(part 1 of 2)
# Autodesk Inventor assembly: Table
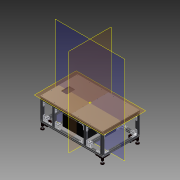
[picture p0: Inventor's stored thumbnail of the model, 180x180]
Saved by Autodesk Inventor 2015 (Build 190159000, 159)
## iProperties
Created: 2015-12-24
Part Number: Table
Document SubType Name: Assembly
Designer: Ryo
Author: Ryo
## Documents named in this file (11)
- D:\Users\Ryo\Documents\Inventor\motoman_cad\SIA5_TABLE\INVENTOR2015\Table.iam
- D:\Users\Ryo\Documents\Inventor\motoman_table\EFS8-4040-580.ipt
- D:\Users\Ryo\Documents\Inventor\motoman_table\EFS8-4040-305.ipt
- D:\Users\Ryo\Documents\Inventor\motoman_cad\SIA5_TABLE\parts\EFS8-4040-1100.ipt
- D:\Users\Ryo\Documents\Inventor\motoman_cad\SIA5_TABLE\parts\SFK-N19T.ipt
- D:\Users\Ryo\Documents\Inventor\motoman_cad\SIA5_TABLE\INVENTOR2015\board.ipt
- D:\Users\Ryo\Documents\Inventor\motoman_cad\SIA5_TABLE\INVENTOR2015\controller_table.ipt
- D:\Users\Ryo\Documents\Inventor\motoman_cad\SIA5_TABLE\INVENTOR2015\controller.ipt
- D:\Users\Ryo\Documents\Inventor\Content Center Files\R2015\ja-JP\JIS B 1176\JIS B 1176 - M8 x 12.ipt
- D:\Users\Ryo\Documents\Inventor\Content Center Files\R2015\ja-JP\JIS B 1176\JIS B 1176 - M6 x 10.ipt
- D:\Users\Ryo\Documents\Inventor\motoman_cad\SIA5_TABLE\INVENTOR2015\foot_parts.iam
## Components (309 placed, 10 different names)
1. EFS8-4040-580:1 — フラッシュ:63, フラッシュ:64, メイト:70, フラッシュ:82, メイト:81, メイト:85, メイト:89, フラッシュ:86, メイト:91, フラッシュ:114
2. EFS8-4040-580:2 — フラッシュ:43, フラッシュ:44, メイト:44, フラッシュ:47, メイト:47, フラッシュ:49, メイト:51, フラッシュ:83, メイト:83, フラッシュ:89, メイト:95, フラッシュ:119, フラッシュ:122
3. EFS8-4040-580:4 — フラッシュ:16, メイト:26, フラッシュ:17, フラッシュ:18, フラッシュ:20, フラッシュ:54, メイト:62, フラッシュ:77, フラッシュ:78, フラッシュ:98, メイト:114, メイト:116, メイト:133
4. EFS8-4040-580:5 — フラッシュ:74, フラッシュ:75, メイト:73, フラッシュ:76, フラッシュ:95, メイト:108, フラッシュ:96, メイト:109, フラッシュ:101, メイト:119, フラッシュ:102, メイト:121
5. EFS8-4040-580:6 — フラッシュ:1, メイト:14, フラッシュ:2, フラッシュ:3, メイト:15, フラッシュ:4, フラッシュ:13, メイト:20, フラッシュ:15, メイト:24, フラッシュ:74, メイト:112, フラッシュ:100, メイト:117, フラッシュ:116, メイト:308, フラッシュ:118, メイト:309
6. EFS8-4040-580:7 — フラッシュ:68, メイト:72, フラッシュ:76, メイト:135, メイト:138, フラッシュ:111, メイト:140, フラッシュ:112, メイト:142
7. EFS8-4040-580:8 — フラッシュ:45, フラッシュ:46, メイト:45, フラッシュ:48, メイト:49, メイト:58, フラッシュ:52, メイト:74, フラッシュ:90, メイト:98, フラッシュ:91, メイト:100
8. EFS8-4040-305:1 — フラッシュ:18, フラッシュ:19, メイト:27, メイト:63, メイト:64, メイト:66, メイト:101, メイト:104
9. EFS8-4040-305:2 — フラッシュ:5, フラッシュ:6, メイト:16, メイト:18, フラッシュ:11, メイト:21, メイト:105, メイト:107
10. EFS8-4040-305:3 — フラッシュ:20, フラッシュ:21, メイト:28, メイト:34, メイト:36, フラッシュ:104, メイト:125, フラッシュ:105, メイト:128, メイト:134, フラッシュ:108
11. EFS8-4040-305:4 — フラッシュ:28, フラッシュ:29, メイト:32, メイト:42, メイト:46, フラッシュ:61, メイト:69, フラッシュ:62, メイト:90, メイト:94
12. EFS8-4040-305:5 — フラッシュ:7, フラッシュ:8, フラッシュ:9, メイト:17, メイト:22, メイト:25, メイト:120, フラッシュ:103, メイト:124
13. EFS8-4040-305:6 — フラッシュ:24, フラッシュ:25, メイト:30, フラッシュ:45, メイト:57, メイト:59, メイト:60, メイト:79, メイト:87
14. EFS8-4040-305:7 — フラッシュ:26, フラッシュ:27, メイト:31, メイト:50, メイト:52, メイト:54, フラッシュ:59, フラッシュ:60, メイト:68, メイト:78, メイト:82
15. EFS8-4040-305:8 — フラッシュ:22, フラッシュ:23, メイト:29, メイト:38, メイト:39, メイト:48, メイト:129, メイト:132
16. EFS8-4040-1100:1 — フラッシュ:3, メイト:15, フラッシュ:4, フラッシュ:7, フラッシュ:8, フラッシュ:9, メイト:17, フラッシュ:14, メイト:23, メイト:26, フラッシュ:17, フラッシュ:21, メイト:28, フラッシュ:22, フラッシュ:23, メイト:29, フラッシュ:28, フラッシュ:29, メイト:32, フラッシュ:30, メイト:33, メイト:35, フラッシュ:31, フラッシュ:32, メイト:37, フラッシュ:33, メイト:40, フラッシュ:42, メイト:43, フラッシュ:43, フラッシュ:44, フラッシュ:46, メイト:45, メイト:96, メイト:99, フラッシュ:99, メイト:115, メイト:118, フラッシュ:117, フラッシュ:120, メイト:310
17. EFS8-4040-1100:2 — フラッシュ:61, メイト:69, フラッシュ:62, フラッシュ:63, フラッシュ:68, メイト:72, フラッシュ:87, メイト:92, フラッシュ:88, メイト:93, メイト:122, メイト:123, メイト:126, メイト:127, フラッシュ:106, メイト:130, フラッシュ:107, メイト:131, メイト:139, メイト:141, メイト:307
18. EFS8-4040-1100:3 — フラッシュ:59, フラッシュ:60, メイト:68, フラッシュ:64, メイト:70, フラッシュ:75, メイト:73, フラッシュ:80, メイト:77, フラッシュ:81, メイト:80, フラッシュ:84, メイト:84, フラッシュ:85, メイト:88, フラッシュ:92, メイト:102, フラッシュ:93, メイト:103, フラッシュ:94, メイト:106, メイト:110, フラッシュ:109, メイト:136, フラッシュ:110, メイト:137, フラッシュ:113, メイト:313
19. EFS8-4040-1100:4 — フラッシュ:1, メイト:14, フラッシュ:2, フラッシュ:5, フラッシュ:6, メイト:16, フラッシュ:12, メイト:19, フラッシュ:16, フラッシュ:19, メイト:27, フラッシュ:24, フラッシュ:25, メイト:30, フラッシュ:26, フラッシュ:27, メイト:31, メイト:44, メイト:53, フラッシュ:51, メイト:56, フラッシュ:53, メイト:61, フラッシュ:55, メイト:65, フラッシュ:56, フラッシュ:57, メイト:67, フラッシュ:58, メイト:75, フラッシュ:79, メイト:86, メイト:97, フラッシュ:97, メイト:111, メイト:113, フラッシュ:115, フラッシュ:121, メイト:311
20. SFK-N19T:1 — フラッシュ:42, メイト:42, メイト:43, 挿入:1, 挿入:2, メイト:175, メイト:176, メイト:177, メイト:178
21. SFK-N19T:2 — フラッシュ:53, メイト:60, メイト:61, メイト:239, メイト:240, メイト:241, メイト:242, 挿入:15, 挿入:16
22. SFK-N19T:3 — フラッシュ:54, メイト:62, メイト:63, 挿入:79, 挿入:80, メイト:303, メイト:304, メイト:305, メイト:306
23. SFK-N19T:4 — フラッシュ:47, メイト:46, メイト:47, 挿入:5, 挿入:6, メイト:179, メイト:180, メイト:181, メイト:182
24. SFK-N19T:5 — フラッシュ:49, メイト:50, メイト:51, メイト:52, 挿入:7, 挿入:8, 挿入:19, 挿入:20
25. SFK-N19T:6 — メイト:58, フラッシュ:52, メイト:59, メイト:243, メイト:244, メイト:245, メイト:246, 挿入:23, 挿入:24
26. SFK-N19T:7 — フラッシュ:33, メイト:39, メイト:40, メイト:143, メイト:144, メイト:145, メイト:146, メイト:147, メイト:148, メイト:149, メイト:150
27. SFK-N19T:8 — メイト:35, フラッシュ:31, メイト:36, 挿入:45, 挿入:46, 挿入:55, 挿入:56
28. SFK-N19T:9 — フラッシュ:51, メイト:56, メイト:57, メイト:231, メイト:232, メイト:233, メイト:234, メイト:255, メイト:256, メイト:257, メイト:258
29. SFK-N19T:10 — フラッシュ:13, メイト:20, メイト:21, メイト:291, メイト:292, メイト:293, メイト:294, 挿入:115, 挿入:116
30. SFK-N19T:11 — メイト:53, メイト:54, フラッシュ:58, メイト:223, メイト:224, メイト:225, メイト:226, メイト:227, メイト:228, メイト:229, メイト:230
31. SFK-N19T:12 — フラッシュ:48, メイト:48, メイト:49, メイト:155, メイト:156, メイト:157, メイト:158, 挿入:113, 挿入:114
32. SFK-N19T:13 — フラッシュ:32, メイト:37, メイト:38, メイト:151, メイト:152, メイト:153, メイト:154, メイト:275, メイト:276, メイト:277, メイト:278
33. SFK-N19T:14 — フラッシュ:30, メイト:33, メイト:34, 挿入:37, 挿入:38, 挿入:57, 挿入:58
34. SFK-N19T:15 — メイト:18, フラッシュ:11, フラッシュ:12, メイト:19, メイト:287, メイト:288, メイト:289, メイト:290, 挿入:103, 挿入:104
35. SFK-N19T:16 — フラッシュ:15, メイト:24, メイト:25, 挿入:67, 挿入:68, 挿入:75, 挿入:76
36. SFK-N19T:17 — フラッシュ:55, メイト:64, メイト:65, 挿入:77, 挿入:78, 挿入:89, 挿入:90
37. SFK-N19T:18 — フラッシュ:14, メイト:22, メイト:23, 挿入:59, 挿入:60, 挿入:61, 挿入:62
38. SFK-N19T:19 — フラッシュ:56
39. SFK-N19T:20 — フラッシュ:57, メイト:66, メイト:67, 挿入:81, 挿入:82, 挿入:87, 挿入:88
40. board:1 — メイト:307, フラッシュ:113, フラッシュ:114, 挿入:125, 挿入:126, 挿入:127, 挿入:128, 挿入:129, 挿入:130, 挿入:131, 挿入:132, 挿入:133, 挿入:134, 挿入:135, 挿入:136, 挿入:137, 挿入:138, 挿入:139, 挿入:140, 挿入:141, 挿入:142, 挿入:143, 挿入:144, 挿入:145, 挿入:146, メイト:312, フラッシュ:123
41. controller_table:1 — メイト:74, メイト:75, フラッシュ:77, メイト:76
42. controller:1 — メイト:76, フラッシュ:78, フラッシュ:79
43. SFK-N19T:21 — フラッシュ:80, メイト:77, メイト:78, メイト:219, メイト:220, メイト:221, メイト:222, メイト:263, メイト:264, メイト:265, メイト:266
44. SFK-N19T:22 — フラッシュ:95, メイト:107, メイト:108, メイト:295, メイト:296, メイト:297, メイト:298, 挿入:123, 挿入:124
45. SFK-N19T:23 — フラッシュ:82, メイト:81, メイト:82, 挿入:17, 挿入:18, メイト:267, メイト:268, メイト:269, メイト:270
46. SFK-N19T:24 — フラッシュ:81, メイト:79, メイト:80, メイト:259, メイト:260, メイト:261, メイト:262, 挿入:25, 挿入:26
47. SFK-N19T:25 — フラッシュ:84, メイト:84, メイト:85, 挿入:13, 挿入:14, メイト:247, メイト:248, メイト:249, メイト:250
48. SFK-N19T:26 — フラッシュ:89, メイト:95, メイト:96, メイト:171, メイト:172, メイト:173, メイト:174, メイト:183, メイト:184, メイト:185, メイト:186
49. SFK-N19T:27 — フラッシュ:96, メイト:109, メイト:110, 挿入:99, 挿入:100, 挿入:117, 挿入:118
50. SFK-N19T:28 — フラッシュ:94, メイト:105, メイト:106, 挿入:97, 挿入:98, 挿入:101, 挿入:102
51. SFK-N19T:29 — フラッシュ:88, メイト:93, メイト:94, メイト:195, メイト:196, メイト:197, メイト:198, 挿入:33, 挿入:34
52. SFK-N19T:30 — メイト:89, フラッシュ:86, メイト:90, メイト:199, メイト:200, メイト:201, メイト:202, 挿入:29, 挿入:30
53. SFK-N19T:31 — フラッシュ:93, メイト:103, メイト:104, 挿入:91, 挿入:92, 挿入:93, 挿入:94
54. SFK-N19T:32 — フラッシュ:83, メイト:83, メイト:86, メイト:235, メイト:236, メイト:237, メイト:238, 挿入:21, 挿入:22
55. SFK-N19T:33 — フラッシュ:85, メイト:87, メイト:88, メイト:215, メイト:216, メイト:217, メイト:218, メイト:314, メイト:315, メイト:316, メイト:317
56. SFK-N19T:34 — フラッシュ:87, メイト:91, メイト:92, メイト:187, メイト:188, メイト:189, メイト:190, メイト:191, メイト:192, メイト:193, メイト:194
57. SFK-N19T:35 — フラッシュ:90, メイト:97, メイト:98, メイト:163, メイト:164, メイト:165, メイト:166, メイト:251, メイト:252, メイト:253, メイト:254
58. SFK-N19T:36 — フラッシュ:91, メイト:99, メイト:100, 挿入:3, 挿入:4, メイト:167, メイト:168, メイト:169, メイト:170
59. SFK-N19T:37 — フラッシュ:92, メイト:101, メイト:102, 挿入:83, 挿入:84, 挿入:95, 挿入:96
60. SFK-N19T:38 — フラッシュ:106, メイト:129, メイト:130, 挿入:9, 挿入:10, メイト:271, メイト:272, メイト:273, メイト:274
61. SFK-N19T:39 — フラッシュ:101, メイト:119, メイト:120, 挿入:69, 挿入:70, 挿入:71, 挿入:72
62. SFK-N19T:40 — フラッシュ:103, メイト:123, メイト:124, 挿入:49, 挿入:50, 挿入:51, 挿入:52
63. SFK-N19T:43 — メイト:139, フラッシュ:111, メイト:140, メイト:203, メイト:204, メイト:205, メイト:206, メイト:207, メイト:208, メイト:209, メイト:210
64. SFK-N19T:44 — フラッシュ:109, メイト:135, メイト:136, メイト:211, メイト:212, メイト:213, メイト:214, 挿入:119, 挿入:120
65. SFK-N19T:45 — フラッシュ:107, メイト:131, メイト:132, メイト:159, メイト:160, メイト:161, メイト:162, 挿入:31, 挿入:32
66. SFK-N19T:46 — フラッシュ:104, メイト:125, メイト:126, 挿入:39, 挿入:40, 挿入:41, 挿入:42
67. SFK-N19T:47 — フラッシュ:99, メイト:115, メイト:116, 挿入:43, 挿入:44, 挿入:65, 挿入:66
68. SFK-N19T:48 — フラッシュ:97, メイト:111, メイト:112, 挿入:105, 挿入:106, 挿入:107, 挿入:108
69. SFK-N19T:49 — フラッシュ:105, メイト:127, メイト:128, 挿入:35, 挿入:36, 挿入:47, 挿入:48
70. SFK-N19T:50 — フラッシュ:110, メイト:137, メイト:138, 挿入:27, 挿入:28, 挿入:121, 挿入:122
71. SFK-N19T:51 — メイト:133, メイト:134, フラッシュ:108, 挿入:63, 挿入:64, メイト:279, メイト:280, メイト:281, メイト:282
72. SFK-N19T:52 — フラッシュ:102, メイト:121, メイト:122, 挿入:73, 挿入:74, 挿入:111, 挿入:112
73. SFK-N19T:53 — フラッシュ:98, メイト:113, メイト:114, 挿入:85, 挿入:86, メイト:299, メイト:300, メイト:301, メイト:302
74. SFK-N19T:55 — フラッシュ:100, メイト:117, メイト:118, メイト:283, メイト:284, メイト:285, メイト:286, 挿入:109, 挿入:110
75. SFK-N19T:56 — フラッシュ:112, メイト:141, メイト:142, 挿入:11, 挿入:12, 挿入:53, 挿入:54
76. JIS B 1176 - メートル M8 x 12:1 — メイト:143, メイト:144
77. JIS B 1176 - メートル M8 x 12:2 — メイト:145, メイト:146
78. JIS B 1176 - メートル M8 x 12:3 — 挿入:1
79. JIS B 1176 - メートル M8 x 12:4 — 挿入:2
80. JIS B 1176 - メートル M8 x 12:5 — メイト:147, メイト:148
81. JIS B 1176 - メートル M8 x 12:6 — メイト:149, メイト:150
82. JIS B 1176 - メートル M8 x 12:7 — メイト:151, メイト:152
83. JIS B 1176 - メートル M8 x 12:8 — メイト:153, メイト:154
84. JIS B 1176 - メートル M8 x 12:9 — メイト:155, メイト:156
85. JIS B 1176 - メートル M8 x 12:10 — メイト:157, メイト:158
86. JIS B 1176 - メートル M8 x 12:11 — 挿入:3
87. JIS B 1176 - メートル M8 x 12:12 — 挿入:4
88. JIS B 1176 - メートル M8 x 12:13 — メイト:159, メイト:160
89. JIS B 1176 - メートル M8 x 12:14 — メイト:161, メイト:162
90. JIS B 1176 - メートル M8 x 12:15 — 挿入:5
91. JIS B 1176 - メートル M8 x 12:16 — 挿入:6
92. JIS B 1176 - メートル M8 x 12:17 — メイト:163, メイト:164
93. JIS B 1176 - メートル M8 x 12:18 — メイト:165, メイト:166
94. JIS B 1176 - メートル M8 x 12:19 — 挿入:7
95. JIS B 1176 - メートル M8 x 12:20 — 挿入:8
96. JIS B 1176 - メートル M8 x 12:21 — メイト:167, メイト:168
97. JIS B 1176 - メートル M8 x 12:22 — メイト:169, メイト:170
98. JIS B 1176 - メートル M8 x 12:23 — メイト:171, メイト:172
99. JIS B 1176 - メートル M8 x 12:24 — メイト:173, メイト:174
100. JIS B 1176 - メートル M8 x 12:25 — メイト:175, メイト:176
101. JIS B 1176 - メートル M8 x 12:26 — メイト:177, メイト:178
102. JIS B 1176 - メートル M8 x 12:27 — メイト:179, メイト:180
103. JIS B 1176 - メートル M8 x 12:28 — メイト:181, メイト:182
104. JIS B 1176 - メートル M8 x 12:29 — メイト:183, メイト:184
105. JIS B 1176 - メートル M8 x 12:30 — メイト:185, メイト:186
106. JIS B 1176 - メートル M8 x 12:31 — メイト:187, メイト:188
107. JIS B 1176 - メートル M8 x 12:32 — メイト:189, メイト:190
108. JIS B 1176 - メートル M8 x 12:33 — メイト:191, メイト:192
109. JIS B 1176 - メートル M8 x 12:34 — メイト:193, メイト:194
110. JIS B 1176 - メートル M8 x 12:35 — メイト:195, メイト:196
111. JIS B 1176 - メートル M8 x 12:36 — メイト:197, メイト:198
112. JIS B 1176 - メートル M8 x 12:37 — メイト:199, メイト:200
113. JIS B 1176 - メートル M8 x 12:38 — メイト:201, メイト:202
114. JIS B 1176 - メートル M8 x 12:39 — 挿入:9
115. JIS B 1176 - メートル M8 x 12:40 — 挿入:10
116. JIS B 1176 - メートル M8 x 12:41 — 挿入:11
117. JIS B 1176 - メートル M8 x 12:42 — 挿入:12
118. JIS B 1176 - メートル M8 x 12:43 — メイト:203, メイト:204
119. JIS B 1176 - メートル M8 x 12:44 — メイト:205, メイト:206
120. JIS B 1176 - メートル M8 x 12:45 — メイト:207, メイト:208
121. JIS B 1176 - メートル M8 x 12:46 — メイト:209, メイト:210
122. JIS B 1176 - メートル M8 x 12:47 — メイト:211, メイト:212
123. JIS B 1176 - メートル M8 x 12:48 — メイト:213, メイト:214
124. JIS B 1176 - メートル M8 x 12:49 — 挿入:13
125. JIS B 1176 - メートル M8 x 12:50 — 挿入:14
126. JIS B 1176 - メートル M8 x 12:51 — メイト:215, メイト:216
127. JIS B 1176 - メートル M8 x 12:52 — メイト:217, メイト:218
128. JIS B 1176 - メートル M8 x 12:53 — メイト:219, メイト:220
129. JIS B 1176 - メートル M8 x 12:54 — メイト:221, メイト:222
130. JIS B 1176 - メートル M8 x 12:55 — メイト:223, メイト:224
131. JIS B 1176 - メートル M8 x 12:56 — メイト:225, メイト:226
132. JIS B 1176 - メートル M8 x 12:57 — メイト:227, メイト:228
133. JIS B 1176 - メートル M8 x 12:58 — メイト:229, メイト:230
134. JIS B 1176 - メートル M8 x 12:59 — メイト:231, メイト:232
135. JIS B 1176 - メートル M8 x 12:60 — メイト:233, メイト:234
136. JIS B 1176 - メートル M8 x 12:61 — メイト:235, メイト:236
137. JIS B 1176 - メートル M8 x 12:62 — メイト:237, メイト:238
138. JIS B 1176 - メートル M8 x 12:63 — メイト:239, メイト:240
139. JIS B 1176 - メートル M8 x 12:64 — メイト:241, メイト:242
140. JIS B 1176 - メートル M8 x 12:65 — メイト:243, メイト:244
141. JIS B 1176 - メートル M8 x 12:66 — メイト:245, メイト:246
142. JIS B 1176 - メートル M8 x 12:67 — 挿入:15
143. JIS B 1176 - メートル M8 x 12:68 — 挿入:16
144. JIS B 1176 - メートル M8 x 12:69 — 挿入:17
145. JIS B 1176 - メートル M8 x 12:70 — 挿入:18
146. JIS B 1176 - メートル M8 x 12:71 — メイト:247, メイト:248
147. JIS B 1176 - メートル M8 x 12:72 — メイト:249, メイト:250
148. JIS B 1176 - メートル M8 x 12:73 — 挿入:19
149. JIS B 1176 - メートル M8 x 12:74 — 挿入:20
150. JIS B 1176 - メートル M8 x 12:75 — 挿入:21
151. JIS B 1176 - メートル M8 x 12:76 — 挿入:22
152. JIS B 1176 - メートル M8 x 12:77 — メイト:251, メイト:252
153. JIS B 1176 - メートル M8 x 12:78 — メイト:253, メイト:254
154. JIS B 1176 - メートル M8 x 12:79 — 挿入:23
155. JIS B 1176 - メートル M8 x 12:80 — 挿入:24
156. JIS B 1176 - メートル M8 x 12:81 — メイト:255, メイト:256
157. JIS B 1176 - メートル M8 x 12:82 — メイト:257, メイト:258
158. JIS B 1176 - メートル M8 x 12:83 — メイト:259, メイト:260
159. JIS B 1176 - メートル M8 x 12:84 — メイト:261, メイト:262
160. JIS B 1176 - メートル M8 x 12:85 — 挿入:25
161. JIS B 1176 - メートル M8 x 12:86 — 挿入:26
162. JIS B 1176 - メートル M8 x 12:87 — メイト:263, メイト:264
163. JIS B 1176 - メートル M8 x 12:88 — メイト:265, メイト:266
164. JIS B 1176 - メートル M8 x 12:89 — メイト:267, メイト:268
165. JIS B 1176 - メートル M8 x 12:90 — メイト:269, メイト:270
166. JIS B 1176 - メートル M8 x 12:91 — 挿入:27
167. JIS B 1176 - メートル M8 x 12:92 — 挿入:28
168. JIS B 1176 - メートル M8 x 12:93 — 挿入:29
169. JIS B 1176 - メートル M8 x 12:94 — 挿入:30
170. JIS B 1176 - メートル M8 x 12:95 — 挿入:31
171. JIS B 1176 - メートル M8 x 12:96 — 挿入:32
172. JIS B 1176 - メートル M8 x 12:97 — 挿入:33
173. JIS B 1176 - メートル M8 x 12:98 — 挿入:34
174. JIS B 1176 - メートル M8 x 12:99 — メイト:271, メイト:272
175. JIS B 1176 - メートル M8 x 12:100 — メイト:273, メイト:274
176. JIS B 1176 - メートル M8 x 12:101 — メイト:275, メイト:276
177. JIS B 1176 - メートル M8 x 12:102 — メイト:277, メイト:278
178. JIS B 1176 - メートル M8 x 12:103 — 挿入:35
179. JIS B 1176 - メートル M8 x 12:104 — 挿入:36
180. JIS B 1176 - メートル M8 x 12:105 — 挿入:37
181. JIS B 1176 - メートル M8 x 12:106 — 挿入:38
182. JIS B 1176 - メートル M8 x 12:107 — 挿入:39
183. JIS B 1176 - メートル M8 x 12:108 — 挿入:40
184. JIS B 1176 - メートル M8 x 12:109 — 挿入:41
185. JIS B 1176 - メートル M8 x 12:110 — 挿入:42
186. JIS B 1176 - メートル M8 x 12:111 — 挿入:43
187. JIS B 1176 - メートル M8 x 12:112 — 挿入:44
188. JIS B 1176 - メートル M8 x 12:113 — 挿入:45
189. JIS B 1176 - メートル M8 x 12:114 — 挿入:46
190. JIS B 1176 - メートル M8 x 12:115 — 挿入:47
191. JIS B 1176 - メートル M8 x 12:116 — 挿入:48
192. JIS B 1176 - メートル M8 x 12:117 — 挿入:49
193. JIS B 1176 - メートル M8 x 12:118 — 挿入:50
194. JIS B 1176 - メートル M8 x 12:119 — 挿入:51
195. JIS B 1176 - メートル M8 x 12:120 — 挿入:52
196. JIS B 1176 - メートル M8 x 12:121 — 挿入:53
197. JIS B 1176 - メートル M8 x 12:122 — 挿入:54
198. JIS B 1176 - メートル M8 x 12:123 — 挿入:55
199. JIS B 1176 - メートル M8 x 12:124 — 挿入:56
200. JIS B 1176 - メートル M8 x 12:125 — 挿入:57
201. JIS B 1176 - メートル M8 x 12:126 — 挿入:58
202. JIS B 1176 - メートル M8 x 12:127 — 挿入:59
203. JIS B 1176 - メートル M8 x 12:128 — 挿入:60
204. JIS B 1176 - メートル M8 x 12:129 — 挿入:61
205. JIS B 1176 - メートル M8 x 12:130 — 挿入:62
206. JIS B 1176 - メートル M8 x 12:131 — 挿入:63
207. JIS B 1176 - メートル M8 x 12:132 — 挿入:64
208. JIS B 1176 - メートル M8 x 12:133 — 挿入:65
209. JIS B 1176 - メートル M8 x 12:134 — 挿入:66
210. JIS B 1176 - メートル M8 x 12:135 — 挿入:67
211. JIS B 1176 - メートル M8 x 12:136 — 挿入:68
212. JIS B 1176 - メートル M8 x 12:137 — 挿入:69
213. JIS B 1176 - メートル M8 x 12:138 — 挿入:70
214. JIS B 1176 - メートル M8 x 12:139 — 挿入:71
215. JIS B 1176 - メートル M8 x 12:140 — 挿入:72
216. JIS B 1176 - メートル M8 x 12:141 — 挿入:73
217. JIS B 1176 - メートル M8 x 12:142 — 挿入:74
218. JIS B 1176 - メートル M8 x 12:143 — メイト:279, メイト:280
219. JIS B 1176 - メートル M8 x 12:144 — メイト:281, メイト:282
220. JIS B 1176 - メートル M8 x 12:145 — 挿入:75
221. JIS B 1176 - メートル M8 x 12:146 — 挿入:76
222. JIS B 1176 - メートル M8 x 12:147 — メイト:283, メイト:284
223. JIS B 1176 - メートル M8 x 12:148 — メイト:285, メイト:286
224. JIS B 1176 - メートル M8 x 12:149 — 挿入:77
225. JIS B 1176 - メートル M8 x 12:150 — 挿入:78
226. JIS B 1176 - メートル M8 x 12:151 — 挿入:79
227. JIS B 1176 - メートル M8 x 12:152 — 挿入:80
228. JIS B 1176 - メートル M8 x 12:153 — 挿入:81
229. JIS B 1176 - メートル M8 x 12:154 — 挿入:82
230. JIS B 1176 - メートル M8 x 12:155 — 挿入:83
231. JIS B 1176 - メートル M8 x 12:156 — 挿入:84
232. JIS B 1176 - メートル M8 x 12:157 — 挿入:85
233. JIS B 1176 - メートル M8 x 12:158 — 挿入:86
234. JIS B 1176 - メートル M8 x 12:159 — 挿入:87
235. JIS B 1176 - メートル M8 x 12:160 — 挿入:88
236. JIS B 1176 - メートル M8 x 12:161 — メイト:287, メイト:288
237. JIS B 1176 - メートル M8 x 12:162 — メイト:289, メイト:290
238. JIS B 1176 - メートル M8 x 12:163 — メイト:291, メイト:292
239. JIS B 1176 - メートル M8 x 12:164 — メイト:293, メイト:294
240. JIS B 1176 - メートル M8 x 12:165 — 挿入:89
241. JIS B 1176 - メートル M8 x 12:166 — 挿入:90
242. JIS B 1176 - メートル M8 x 12:167 — 挿入:91
243. JIS B 1176 - メートル M8 x 12:168 — 挿入:92
244. JIS B 1176 - メートル M8 x 12:169 — 挿入:93
245. JIS B 1176 - メートル M8 x 12:170 — 挿入:94
246. JIS B 1176 - メートル M8 x 12:171 — 挿入:95
247. JIS B 1176 - メートル M8 x 12:172 — 挿入:96
248. JIS B 1176 - メートル M8 x 12:173 — 挿入:97
249. JIS B 1176 - メートル M8 x 12:174 — 挿入:98
250. JIS B 1176 - メートル M8 x 12:175 — 挿入:99
251. JIS B 1176 - メートル M8 x 12:176 — 挿入:100
252. JIS B 1176 - メートル M8 x 12:177 — メイト:295, メイト:296
253. JIS B 1176 - メートル M8 x 12:178 — メイト:297, メイト:298
254. JIS B 1176 - メートル M8 x 12:179 — 挿入:101
255. JIS B 1176 - メートル M8 x 12:180 — 挿入:102
256. JIS B 1176 - メートル M8 x 12:181 — 挿入:103
257. JIS B 1176 - メートル M8 x 12:182 — 挿入:104
258. JIS B 1176 - メートル M8 x 12:183 — 挿入:105
259. JIS B 1176 - メートル M8 x 12:184 — 挿入:106
260. JIS B 1176 - メートル M8 x 12:185 — 挿入:107
261. JIS B 1176 - メートル M8 x 12:186 — 挿入:108
262. JIS B 1176 - メートル M8 x 12:187 — メイト:299, メイト:300
263. JIS B 1176 - メートル M8 x 12:188 — メイト:301, メイト:302
264. JIS B 1176 - メートル M8 x 12:189 — 挿入:109
265. JIS B 1176 - メートル M8 x 12:190 — 挿入:110
266. JIS B 1176 - メートル M8 x 12:191 — 挿入:111
267. JIS B 1176 - メートル M8 x 12:192 — 挿入:112
268. JIS B 1176 - メートル M8 x 12:193 — 挿入:113
269. JIS B 1176 - メートル M8 x 12:194 — 挿入:114
270. JIS B 1176 - メートル M8 x 12:195 — メイト:303, メイト:304
271. JIS B 1176 - メートル M8 x 12:196 — メイト:305, メイト:306
272. JIS B 1176 - メートル M8 x 12:197 — 挿入:115
273. JIS B 1176 - メートル M8 x 12:198 — 挿入:116
274. JIS B 1176 - メートル M8 x 12:199 — 挿入:117
275. JIS B 1176 - メートル M8 x 12:200 — 挿入:118
276. JIS B 1176 - メートル M8 x 12:201 — 挿入:119
277. JIS B 1176 - メートル M8 x 12:202 — 挿入:120
278. JIS B 1176 - メートル M8 x 12:203 — 挿入:121
279. JIS B 1176 - メートル M8 x 12:204 — 挿入:122
280. JIS B 1176 - メートル M8 x 12:205 — 挿入:123
281. JIS B 1176 - メートル M8 x 12:206 — 挿入:124
282. JIS B 1176 - メートル M6 x 10:1 — 挿入:125
283. JIS B 1176 - メートル M6 x 10:2 — 挿入:126
284. JIS B 1176 - メートル M6 x 10:3 — 挿入:127
285. JIS B 1176 - メートル M6 x 10:4 — 挿入:128
286. JIS B 1176 - メートル M6 x 10:5 — 挿入:129
287. JIS B 1176 - メートル M6 x 10:6 — 挿入:130
288. JIS B 1176 - メートル M6 x 10:7 — 挿入:131
289. JIS B 1176 - メートル M6 x 10:8 — 挿入:132
290. JIS B 1176 - メートル M6 x 10:9 — 挿入:133
291. JIS B 1176 - メートル M6 x 10:10 — 挿入:134
292. JIS B 1176 - メートル M6 x 10:11 — 挿入:135
293. JIS B 1176 - メートル M6 x 10:12 — 挿入:136
294. JIS B 1176 - メートル M6 x 10:13 — 挿入:137
295. JIS B 1176 - メートル M6 x 10:14 — 挿入:138
296. JIS B 1176 - メートル M6 x 10:15 — 挿入:139
297. JIS B 1176 - メートル M6 x 10:16 — 挿入:140
298. JIS B 1176 - メートル M6 x 10:17 — 挿入:141
299. JIS B 1176 - メートル M6 x 10:18 — 挿入:142
300. JIS B 1176 - メートル M6 x 10:19 — 挿入:143
301. JIS B 1176 - メートル M6 x 10:20 — 挿入:144
302. JIS B 1176 - メートル M6 x 10:21 — 挿入:145
303. JIS B 1176 - メートル M6 x 10:22 — 挿入:146
304. foot_parts:1 [sub-assembly] — フラッシュ:115, フラッシュ:116, メイト:308
305. foot_parts:2 [sub-assembly] — フラッシュ:117, フラッシュ:118, メイト:309
306. foot_parts:3 [sub-assembly] — フラッシュ:119, フラッシュ:120, メイト:310
307. foot_parts:4 [sub-assembly] — フラッシュ:121, フラッシュ:122, メイト:311
308. JIS B 1176 - メートル M8 x 12:207 — メイト:314, メイト:315
309. JIS B 1176 - メートル M8 x 12:208 — メイト:316, メイト:317
## Relationships (552: Mate 301, Insert 146, Flush 105)
- フラッシュ:1 [Flush]: EFS8-4040-580:6 ↔ EFS8-4040-1100:4
- メイト:14 [Mate]: EFS8-4040-580:6 ↔ EFS8-4040-1100:4
- フラッシュ:2 [Flush]: EFS8-4040-580:6 ↔ EFS8-4040-1100:4
- フラッシュ:3 [Flush]: EFS8-4040-580:6 ↔ EFS8-4040-1100:1
- メイト:15 [Mate]: EFS8-4040-580:6 ↔ EFS8-4040-1100:1
- フラッシュ:4 [Flush]: EFS8-4040-580:6 ↔ EFS8-4040-1100:1
- フラッシュ:5 [Flush]: EFS8-4040-305:2 ↔ EFS8-4040-1100:4
- フラッシュ:6 [Flush]: EFS8-4040-305:2 ↔ EFS8-4040-1100:4
- メイト:16 [Mate]: EFS8-4040-305:2 ↔ EFS8-4040-1100:4
- フラッシュ:7 [Flush]: EFS8-4040-305:5 ↔ EFS8-4040-1100:1
- フラッシュ:8 [Flush]: EFS8-4040-305:5 ↔ EFS8-4040-1100:1
- フラッシュ:9 [Flush]: EFS8-4040-305:5 ↔ EFS8-4040-1100:1
- メイト:17 [Mate]: EFS8-4040-305:5 ↔ EFS8-4040-1100:1
- メイト:18 [Mate]: EFS8-4040-305:2 ↔ SFK-N19T:15
- フラッシュ:11 [Flush] (5 mm): EFS8-4040-305:2 ↔ SFK-N19T:15
- フラッシュ:12 [Flush] (5 mm): EFS8-4040-1100:4 ↔ SFK-N19T:15
- メイト:19 [Mate]: EFS8-4040-1100:4 ↔ SFK-N19T:15
- フラッシュ:13 [Flush] (5 mm): EFS8-4040-580:6 ↔ SFK-N19T:10
- メイト:20 [Mate]: EFS8-4040-580:6 ↔ SFK-N19T:10
- メイト:21 [Mate]: EFS8-4040-305:2 ↔ SFK-N19T:10
- フラッシュ:14 [Flush] (5 mm): EFS8-4040-1100:1 ↔ SFK-N19T:18
- メイト:22 [Mate]: EFS8-4040-305:5 ↔ SFK-N19T:18
- メイト:23 [Mate]: EFS8-4040-1100:1 ↔ SFK-N19T:18
- フラッシュ:15 [Flush] (5 mm): EFS8-4040-580:6 ↔ SFK-N19T:16
- メイト:24 [Mate]: EFS8-4040-580:6 ↔ SFK-N19T:16
- メイト:25 [Mate]: EFS8-4040-305:5 ↔ SFK-N19T:16
- フラッシュ:16 [Flush] (295 mm): EFS8-4040-580:4 ↔ EFS8-4040-1100:4
- メイト:26 [Mate]: EFS8-4040-580:4 ↔ EFS8-4040-1100:1
- フラッシュ:17 [Flush]: EFS8-4040-580:4 ↔ EFS8-4040-1100:1
- フラッシュ:18 [Flush]: EFS8-4040-580:4 ↔ EFS8-4040-305:1
- フラッシュ:19 [Flush]: EFS8-4040-305:1 ↔ EFS8-4040-1100:4
- メイト:27 [Mate]: EFS8-4040-305:1 ↔ EFS8-4040-1100:4
- フラッシュ:20 [Flush]: EFS8-4040-580:4 ↔ EFS8-4040-305:3
- フラッシュ:21 [Flush]: EFS8-4040-305:3 ↔ EFS8-4040-1100:1
- メイト:28 [Mate]: EFS8-4040-305:3 ↔ EFS8-4040-1100:1
- フラッシュ:22 [Flush] (210 mm): EFS8-4040-305:8 ↔ EFS8-4040-1100:1
- フラッシュ:23 [Flush]: EFS8-4040-305:8 ↔ EFS8-4040-1100:1
- メイト:29 [Mate]: EFS8-4040-305:8 ↔ EFS8-4040-1100:1
- フラッシュ:24 [Flush] (210 mm): EFS8-4040-305:6 ↔ EFS8-4040-1100:4
- フラッシュ:25 [Flush]: EFS8-4040-305:6 ↔ EFS8-4040-1100:4
- メイト:30 [Mate]: EFS8-4040-305:6 ↔ EFS8-4040-1100:4
- フラッシュ:26 [Flush]: EFS8-4040-305:7 ↔ EFS8-4040-1100:4
- フラッシュ:27 [Flush]: EFS8-4040-305:7 ↔ EFS8-4040-1100:4
- メイト:31 [Mate]: EFS8-4040-305:7 ↔ EFS8-4040-1100:4
- フラッシュ:28 [Flush]: EFS8-4040-305:4 ↔ EFS8-4040-1100:1
- フラッシュ:29 [Flush]: EFS8-4040-305:4 ↔ EFS8-4040-1100:1
- メイト:32 [Mate]: EFS8-4040-305:4 ↔ EFS8-4040-1100:1
- フラッシュ:30 [Flush] (5 mm): EFS8-4040-1100:1 ↔ SFK-N19T:14
- メイト:33 [Mate]: EFS8-4040-1100:1 ↔ SFK-N19T:14
- メイト:34 [Mate]: EFS8-4040-305:3 ↔ SFK-N19T:14
- メイト:35 [Mate]: EFS8-4040-1100:1 ↔ SFK-N19T:8
- フラッシュ:31 [Flush] (5 mm): EFS8-4040-1100:1 ↔ SFK-N19T:8
- メイト:36 [Mate]: EFS8-4040-305:3 ↔ SFK-N19T:8
- フラッシュ:32 [Flush] (5 mm): EFS8-4040-1100:1 ↔ SFK-N19T:13
- メイト:37 [Mate]: EFS8-4040-1100:1 ↔ SFK-N19T:13
- メイト:38 [Mate]: EFS8-4040-305:8 ↔ SFK-N19T:13
- フラッシュ:33 [Flush] (5 mm): EFS8-4040-1100:1 ↔ SFK-N19T:7
- メイト:39 [Mate]: EFS8-4040-305:8 ↔ SFK-N19T:7
- メイト:40 [Mate]: EFS8-4040-1100:1 ↔ SFK-N19T:7
- フラッシュ:42 [Flush] (5 mm): EFS8-4040-1100:1 ↔ SFK-N19T:1
- メイト:42 [Mate]: EFS8-4040-305:4 ↔ SFK-N19T:1
- メイト:43 [Mate]: EFS8-4040-1100:1 ↔ SFK-N19T:1
- フラッシュ:43 [Flush]: EFS8-4040-580:2 ↔ EFS8-4040-1100:1
- フラッシュ:44 [Flush]: EFS8-4040-580:2 ↔ EFS8-4040-1100:1
- メイト:44 [Mate]: EFS8-4040-580:2 ↔ EFS8-4040-1100:4
- フラッシュ:45 [Flush]: EFS8-4040-580:8 ↔ EFS8-4040-305:6
- フラッシュ:46 [Flush]: EFS8-4040-580:8 ↔ EFS8-4040-1100:1
- メイト:45 [Mate]: EFS8-4040-580:8 ↔ EFS8-4040-1100:1
- フラッシュ:47 [Flush] (5 mm): EFS8-4040-580:2 ↔ SFK-N19T:4
- メイト:46 [Mate]: EFS8-4040-305:4 ↔ SFK-N19T:4
- メイト:47 [Mate]: EFS8-4040-580:2 ↔ SFK-N19T:4
- フラッシュ:48 [Flush] (5 mm): EFS8-4040-580:8 ↔ SFK-N19T:12
- メイト:48 [Mate]: EFS8-4040-305:8 ↔ SFK-N19T:12
- メイト:49 [Mate]: EFS8-4040-580:8 ↔ SFK-N19T:12
- フラッシュ:49 [Flush] (5 mm): EFS8-4040-580:2 ↔ SFK-N19T:5
- メイト:50 [Mate]: EFS8-4040-305:7 ↔ SFK-N19T:5
- メイト:51 [Mate]: EFS8-4040-580:2 ↔ SFK-N19T:5
- メイト:52 [Mate]: EFS8-4040-305:7 ↔ SFK-N19T:5
- メイト:53 [Mate]: EFS8-4040-1100:4 ↔ SFK-N19T:11
- メイト:54 [Mate]: EFS8-4040-305:7 ↔ SFK-N19T:11
- フラッシュ:51 [Flush] (5 mm): EFS8-4040-1100:4 ↔ SFK-N19T:9
- メイト:56 [Mate]: EFS8-4040-1100:4 ↔ SFK-N19T:9
- メイト:57 [Mate]: EFS8-4040-305:6 ↔ SFK-N19T:9
- メイト:58 [Mate]: EFS8-4040-580:8 ↔ SFK-N19T:6
- フラッシュ:52 [Flush] (5 mm): EFS8-4040-580:8 ↔ SFK-N19T:6
- メイト:59 [Mate]: EFS8-4040-305:6 ↔ SFK-N19T:6
- フラッシュ:53 [Flush] (5 mm): EFS8-4040-1100:4 ↔ SFK-N19T:2
- メイト:60 [Mate]: EFS8-4040-305:6 ↔ SFK-N19T:2
- メイト:61 [Mate]: EFS8-4040-1100:4 ↔ SFK-N19T:2
- フラッシュ:54 [Flush] (5 mm): EFS8-4040-580:4 ↔ SFK-N19T:3
- メイト:62 [Mate]: EFS8-4040-580:4 ↔ SFK-N19T:3
- メイト:63 [Mate]: EFS8-4040-305:1 ↔ SFK-N19T:3
- フラッシュ:55 [Flush] (5 mm): EFS8-4040-1100:4 ↔ SFK-N19T:17
- メイト:64 [Mate]: EFS8-4040-305:1 ↔ SFK-N19T:17
- メイト:65 [Mate]: EFS8-4040-1100:4 ↔ SFK-N19T:17
- フラッシュ:56 [Flush] (5 mm): EFS8-4040-1100:4 ↔ SFK-N19T:19
- フラッシュ:57 [Flush] (5 mm): EFS8-4040-1100:4 ↔ SFK-N19T:20
- メイト:66 [Mate]: EFS8-4040-305:1 ↔ SFK-N19T:20
- メイト:67 [Mate]: EFS8-4040-1100:4 ↔ SFK-N19T:20
- フラッシュ:58 [Flush] (5 mm): EFS8-4040-1100:4 ↔ SFK-N19T:11
- フラッシュ:59 [Flush]: EFS8-4040-305:7 ↔ EFS8-4040-1100:3
- フラッシュ:60 [Flush]: EFS8-4040-305:7 ↔ EFS8-4040-1100:3
- メイト:68 [Mate]: EFS8-4040-305:7 ↔ EFS8-4040-1100:3
- フラッシュ:61 [Flush]: EFS8-4040-305:4 ↔ EFS8-4040-1100:2
- メイト:69 [Mate]: EFS8-4040-305:4 ↔ EFS8-4040-1100:2
- フラッシュ:62 [Flush]: EFS8-4040-305:4 ↔ EFS8-4040-1100:2
- フラッシュ:63 [Flush]: EFS8-4040-580:1 ↔ EFS8-4040-1100:2
- フラッシュ:64 [Flush]: EFS8-4040-580:1 ↔ EFS8-4040-1100:3
- メイト:70 [Mate]: EFS8-4040-580:1 ↔ EFS8-4040-1100:3
- フラッシュ:68 [Flush]: EFS8-4040-580:7 ↔ EFS8-4040-1100:2
- メイト:72 [Mate]: EFS8-4040-580:7 ↔ EFS8-4040-1100:2
- フラッシュ:74 [Flush]: EFS8-4040-580:5 ↔ EFS8-4040-580:6
- フラッシュ:75 [Flush]: EFS8-4040-580:5 ↔ EFS8-4040-1100:3
- メイト:73 [Mate]: EFS8-4040-580:5 ↔ EFS8-4040-1100:3
- フラッシュ:76 [Flush] (530 mm): EFS8-4040-580:5 ↔ EFS8-4040-580:7
- メイト:74 [Mate]: EFS8-4040-580:8 ↔ controller_table:1
- メイト:75 [Mate]: EFS8-4040-1100:4 ↔ controller_table:1
- フラッシュ:77 [Flush]: EFS8-4040-580:4 ↔ controller_table:1
- メイト:76 [Mate]: controller_table:1 ↔ controller:1
- フラッシュ:78 [Flush] (-87.5 mm): EFS8-4040-580:4 ↔ controller:1
- フラッシュ:79 [Flush] (95 mm): EFS8-4040-1100:4 ↔ controller:1
- フラッシュ:80 [Flush] (5 mm): EFS8-4040-1100:3 ↔ SFK-N19T:21
- メイト:77 [Mate]: EFS8-4040-1100:3 ↔ SFK-N19T:21
- メイト:78 [Mate]: EFS8-4040-305:7 ↔ SFK-N19T:21
- フラッシュ:81 [Flush] (5 mm): EFS8-4040-1100:3 ↔ SFK-N19T:24
- メイト:79 [Mate]: EFS8-4040-305:6 ↔ SFK-N19T:24
- メイト:80 [Mate]: EFS8-4040-1100:3 ↔ SFK-N19T:24
- フラッシュ:82 [Flush] (5 mm): EFS8-4040-580:1 ↔ SFK-N19T:23
- メイト:81 [Mate]: EFS8-4040-580:1 ↔ SFK-N19T:23
- メイト:82 [Mate]: EFS8-4040-305:7 ↔ SFK-N19T:23
- フラッシュ:83 [Flush] (5 mm): EFS8-4040-580:2 ↔ SFK-N19T:32
- メイト:83 [Mate]: EFS8-4040-580:2 ↔ SFK-N19T:32
- フラッシュ:84 [Flush] (5 mm): EFS8-4040-1100:3 ↔ SFK-N19T:25
- メイト:84 [Mate]: EFS8-4040-1100:3 ↔ SFK-N19T:25
- メイト:85 [Mate]: EFS8-4040-580:1 ↔ SFK-N19T:25
- メイト:86 [Mate]: EFS8-4040-1100:4 ↔ SFK-N19T:32
- フラッシュ:85 [Flush] (5 mm): EFS8-4040-1100:3 ↔ SFK-N19T:33
- メイト:87 [Mate]: EFS8-4040-305:6 ↔ SFK-N19T:33
- メイト:88 [Mate]: EFS8-4040-1100:3 ↔ SFK-N19T:33
- メイト:89 [Mate]: EFS8-4040-580:1 ↔ SFK-N19T:30
- フラッシュ:86 [Flush] (5 mm): EFS8-4040-580:1 ↔ SFK-N19T:30
- メイト:90 [Mate]: EFS8-4040-305:4 ↔ SFK-N19T:30
- フラッシュ:87 [Flush] (5 mm): EFS8-4040-1100:2 ↔ SFK-N19T:34
- メイト:91 [Mate]: EFS8-4040-580:1 ↔ SFK-N19T:34
- メイト:92 [Mate]: EFS8-4040-1100:2 ↔ SFK-N19T:34
- フラッシュ:88 [Flush] (5 mm): EFS8-4040-1100:2 ↔ SFK-N19T:29
- メイト:93 [Mate]: EFS8-4040-1100:2 ↔ SFK-N19T:29
- メイト:94 [Mate]: EFS8-4040-305:4 ↔ SFK-N19T:29
- フラッシュ:89 [Flush] (5 mm): EFS8-4040-580:2 ↔ SFK-N19T:26
- メイト:95 [Mate]: EFS8-4040-580:2 ↔ SFK-N19T:26
- メイト:96 [Mate]: EFS8-4040-1100:1 ↔ SFK-N19T:26
- フラッシュ:90 [Flush] (5 mm): EFS8-4040-580:8 ↔ SFK-N19T:35
- メイト:97 [Mate]: EFS8-4040-1100:4 ↔ SFK-N19T:35
- メイト:98 [Mate]: EFS8-4040-580:8 ↔ SFK-N19T:35
- フラッシュ:91 [Flush] (5 mm): EFS8-4040-580:8 ↔ SFK-N19T:36
- メイト:99 [Mate]: EFS8-4040-1100:1 ↔ SFK-N19T:36
- メイト:100 [Mate]: EFS8-4040-580:8 ↔ SFK-N19T:36
- フラッシュ:92 [Flush] (5 mm): EFS8-4040-1100:3 ↔ SFK-N19T:37
- メイト:101 [Mate]: EFS8-4040-305:1 ↔ SFK-N19T:37
- メイト:102 [Mate]: EFS8-4040-1100:3 ↔ SFK-N19T:37
- フラッシュ:93 [Flush]: EFS8-4040-1100:3 ↔ SFK-N19T:31
- メイト:103 [Mate]: EFS8-4040-1100:3 ↔ SFK-N19T:31
- メイト:104 [Mate]: EFS8-4040-305:1 ↔ SFK-N19T:31
- フラッシュ:94 [Flush] (5 mm): EFS8-4040-1100:3 ↔ SFK-N19T:28
- メイト:105 [Mate]: EFS8-4040-305:2 ↔ SFK-N19T:28
- メイト:106 [Mate]: EFS8-4040-1100:3 ↔ SFK-N19T:28
- フラッシュ:95 [Flush] (5 mm): EFS8-4040-580:5 ↔ SFK-N19T:22
- メイト:107 [Mate]: EFS8-4040-305:2 ↔ SFK-N19T:22
- メイト:108 [Mate]: EFS8-4040-580:5 ↔ SFK-N19T:22
- フラッシュ:96 [Flush]: EFS8-4040-580:5 ↔ SFK-N19T:27
- メイト:109 [Mate]: EFS8-4040-580:5 ↔ SFK-N19T:27
- メイト:110 [Mate]: EFS8-4040-1100:3 ↔ SFK-N19T:27
- フラッシュ:97 [Flush] (5 mm): EFS8-4040-1100:4 ↔ SFK-N19T:48
- メイト:111 [Mate]: EFS8-4040-1100:4 ↔ SFK-N19T:48
- メイト:112 [Mate]: EFS8-4040-580:6 ↔ SFK-N19T:48
- フラッシュ:98 [Flush] (5 mm): EFS8-4040-580:4 ↔ SFK-N19T:53
- メイト:113 [Mate]: EFS8-4040-1100:4 ↔ SFK-N19T:53
- メイト:114 [Mate]: EFS8-4040-580:4 ↔ SFK-N19T:53
- フラッシュ:99 [Flush] (5 mm): EFS8-4040-1100:1 ↔ SFK-N19T:47
- メイト:115 [Mate]: EFS8-4040-1100:1 ↔ SFK-N19T:47
- メイト:116 [Mate]: EFS8-4040-580:4 ↔ SFK-N19T:47
- フラッシュ:100 [Flush] (5 mm): EFS8-4040-580:6 ↔ SFK-N19T:55
- メイト:117 [Mate]: EFS8-4040-580:6 ↔ SFK-N19T:55
- メイト:118 [Mate]: EFS8-4040-1100:1 ↔ SFK-N19T:55
- フラッシュ:101 [Flush] (5 mm): EFS8-4040-580:5 ↔ SFK-N19T:39
- メイト:119 [Mate]: EFS8-4040-580:5 ↔ SFK-N19T:39
- メイト:120 [Mate]: EFS8-4040-305:5 ↔ SFK-N19T:39
- フラッシュ:102 [Flush] (5 mm): EFS8-4040-580:5 ↔ SFK-N19T:52
- メイト:121 [Mate]: EFS8-4040-580:5 ↔ SFK-N19T:52
- メイト:122 [Mate]: EFS8-4040-1100:2 ↔ SFK-N19T:52
- フラッシュ:103 [Flush]: EFS8-4040-305:5 ↔ SFK-N19T:40
- メイト:123 [Mate]: EFS8-4040-1100:2 ↔ SFK-N19T:40
- メイト:124 [Mate]: EFS8-4040-305:5 ↔ SFK-N19T:40
- フラッシュ:104 [Flush]: EFS8-4040-305:3 ↔ SFK-N19T:46
- メイト:125 [Mate]: EFS8-4040-305:3 ↔ SFK-N19T:46
- メイト:126 [Mate]: EFS8-4040-1100:2 ↔ SFK-N19T:46
- フラッシュ:105 [Flush] (5 mm): EFS8-4040-305:3 ↔ SFK-N19T:49
- メイト:127 [Mate]: EFS8-4040-1100:2 ↔ SFK-N19T:49
- メイト:128 [Mate]: EFS8-4040-305:3 ↔ SFK-N19T:49
- フラッシュ:106 [Flush] (5 mm): EFS8-4040-1100:2 ↔ SFK-N19T:38
- メイト:129 [Mate]: EFS8-4040-305:8 ↔ SFK-N19T:38
- メイト:130 [Mate]: EFS8-4040-1100:2 ↔ SFK-N19T:38
- フラッシュ:107 [Flush] (5 mm): EFS8-4040-1100:2 ↔ SFK-N19T:45
- メイト:131 [Mate]: EFS8-4040-1100:2 ↔ SFK-N19T:45
- メイト:132 [Mate]: EFS8-4040-305:8 ↔ SFK-N19T:45
- メイト:133 [Mate]: EFS8-4040-580:4 ↔ SFK-N19T:51
- メイト:134 [Mate]: EFS8-4040-305:3 ↔ SFK-N19T:51
- フラッシュ:108 [Flush] (5 mm): EFS8-4040-305:3 ↔ SFK-N19T:51
- フラッシュ:109 [Flush] (5 mm): EFS8-4040-1100:3 ↔ SFK-N19T:44
- メイト:135 [Mate]: EFS8-4040-580:7 ↔ SFK-N19T:44
- メイト:136 [Mate]: EFS8-4040-1100:3 ↔ SFK-N19T:44
- フラッシュ:110 [Flush] (5 mm): EFS8-4040-1100:3 ↔ SFK-N19T:50
- メイト:137 [Mate]: EFS8-4040-1100:3 ↔ SFK-N19T:50
- メイト:138 [Mate]: EFS8-4040-580:7 ↔ SFK-N19T:50
- メイト:139 [Mate]: EFS8-4040-1100:2 ↔ SFK-N19T:43
- フラッシュ:111 [Flush] (5 mm): EFS8-4040-580:7 ↔ SFK-N19T:43
- メイト:140 [Mate]: EFS8-4040-580:7 ↔ SFK-N19T:43
- フラッシュ:112 [Flush] (5 mm): EFS8-4040-580:7 ↔ SFK-N19T:56
- メイト:141 [Mate]: EFS8-4040-1100:2 ↔ SFK-N19T:56
- メイト:142 [Mate]: EFS8-4040-580:7 ↔ SFK-N19T:56
- メイト:143 [Mate]: SFK-N19T:7 ↔ JIS B 1176 - メートル M8 x 12:1
- メイト:144 [Mate]: SFK-N19T:7 ↔ JIS B 1176 - メートル M8 x 12:1
- メイト:145 [Mate]: SFK-N19T:7 ↔ JIS B 1176 - メートル M8 x 12:2
- メイト:146 [Mate]: SFK-N19T:7 ↔ JIS B 1176 - メートル M8 x 12:2
- 挿入:1 [Insert]: SFK-N19T:1 ↔ JIS B 1176 - メートル M8 x 12:3
- 挿入:2 [Insert]: SFK-N19T:1 ↔ JIS B 1176 - メートル M8 x 12:4
- メイト:147 [Mate]: SFK-N19T:7 ↔ JIS B 1176 - メートル M8 x 12:5
- メイト:148 [Mate]: SFK-N19T:7 ↔ JIS B 1176 - メートル M8 x 12:5
- メイト:149 [Mate]: SFK-N19T:7 ↔ JIS B 1176 - メートル M8 x 12:6
- メイト:150 [Mate]: SFK-N19T:7 ↔ JIS B 1176 - メートル M8 x 12:6
- メイト:151 [Mate]: SFK-N19T:13 ↔ JIS B 1176 - メートル M8 x 12:7
- メイト:152 [Mate]: SFK-N19T:13 ↔ JIS B 1176 - メートル M8 x 12:7
- メイト:153 [Mate]: SFK-N19T:13 ↔ JIS B 1176 - メートル M8 x 12:8
- メイト:154 [Mate]: SFK-N19T:13 ↔ JIS B 1176 - メートル M8 x 12:8
- メイト:155 [Mate]: SFK-N19T:12 ↔ JIS B 1176 - メートル M8 x 12:9
- メイト:156 [Mate]: SFK-N19T:12 ↔ JIS B 1176 - メートル M8 x 12:9
- メイト:157 [Mate]: SFK-N19T:12 ↔ JIS B 1176 - メートル M8 x 12:10
- メイト:158 [Mate]: SFK-N19T:12 ↔ JIS B 1176 - メートル M8 x 12:10
- 挿入:3 [Insert]: SFK-N19T:36 ↔ JIS B 1176 - メートル M8 x 12:11
- 挿入:4 [Insert]: SFK-N19T:36 ↔ JIS B 1176 - メートル M8 x 12:12
- メイト:159 [Mate]: SFK-N19T:45 ↔ JIS B 1176 - メートル M8 x 12:13
- メイト:160 [Mate]: SFK-N19T:45 ↔ JIS B 1176 - メートル M8 x 12:13
- メイト:161 [Mate]: SFK-N19T:45 ↔ JIS B 1176 - メートル M8 x 12:14
- メイト:162 [Mate]: SFK-N19T:45 ↔ JIS B 1176 - メートル M8 x 12:14
- 挿入:5 [Insert]: SFK-N19T:4 ↔ JIS B 1176 - メートル M8 x 12:15
- 挿入:6 [Insert]: SFK-N19T:4 ↔ JIS B 1176 - メートル M8 x 12:16
- メイト:163 [Mate]: SFK-N19T:35 ↔ JIS B 1176 - メートル M8 x 12:17
- メイト:164 [Mate]: SFK-N19T:35 ↔ JIS B 1176 - メートル M8 x 12:17
- メイト:165 [Mate]: SFK-N19T:35 ↔ JIS B 1176 - メートル M8 x 12:18
- メイト:166 [Mate]: SFK-N19T:35 ↔ JIS B 1176 - メートル M8 x 12:18
- 挿入:7 [Insert]: SFK-N19T:5 ↔ JIS B 1176 - メートル M8 x 12:19
- 挿入:8 [Insert]: SFK-N19T:5 ↔ JIS B 1176 - メートル M8 x 12:20
- メイト:167 [Mate]: SFK-N19T:36 ↔ JIS B 1176 - メートル M8 x 12:21
- メイト:168 [Mate]: SFK-N19T:36 ↔ JIS B 1176 - メートル M8 x 12:21
- メイト:169 [Mate]: SFK-N19T:36 ↔ JIS B 1176 - メートル M8 x 12:22
- メイト:170 [Mate]: SFK-N19T:36 ↔ JIS B 1176 - メートル M8 x 12:22
- メイト:171 [Mate]: SFK-N19T:26 ↔ JIS B 1176 - メートル M8 x 12:23
- メイト:172 [Mate]: SFK-N19T:26 ↔ JIS B 1176 - メートル M8 x 12:23
- メイト:173 [Mate]: SFK-N19T:26 ↔ JIS B 1176 - メートル M8 x 12:24
- メイト:174 [Mate]: SFK-N19T:26 ↔ JIS B 1176 - メートル M8 x 12:24
- メイト:175 [Mate]: SFK-N19T:1 ↔ JIS B 1176 - メートル M8 x 12:25
- メイト:176 [Mate]: SFK-N19T:1 ↔ JIS B 1176 - メートル M8 x 12:25
- メイト:177 [Mate]: SFK-N19T:1 ↔ JIS B 1176 - メートル M8 x 12:26
- メイト:178 [Mate]: SFK-N19T:1 ↔ JIS B 1176 - メートル M8 x 12:26
- メイト:179 [Mate]: SFK-N19T:4 ↔ JIS B 1176 - メートル M8 x 12:27
- メイト:180 [Mate]: SFK-N19T:4 ↔ JIS B 1176 - メートル M8 x 12:27
- メイト:181 [Mate]: SFK-N19T:4 ↔ JIS B 1176 - メートル M8 x 12:28
- メイト:182 [Mate]: SFK-N19T:4 ↔ JIS B 1176 - メートル M8 x 12:28
- メイト:183 [Mate]: SFK-N19T:26 ↔ JIS B 1176 - メートル M8 x 12:29
- メイト:184 [Mate]: SFK-N19T:26 ↔ JIS B 1176 - メートル M8 x 12:29
- メイト:185 [Mate]: SFK-N19T:26 ↔ JIS B 1176 - メートル M8 x 12:30
- メイト:186 [Mate]: SFK-N19T:26 ↔ JIS B 1176 - メートル M8 x 12:30
- メイト:187 [Mate]: SFK-N19T:34 ↔ JIS B 1176 - メートル M8 x 12:31
- メイト:188 [Mate]: SFK-N19T:34 ↔ JIS B 1176 - メートル M8 x 12:31
- メイト:189 [Mate]: SFK-N19T:34 ↔ JIS B 1176 - メートル M8 x 12:32
- メイト:190 [Mate]: SFK-N19T:34 ↔ JIS B 1176 - メートル M8 x 12:32
- メイト:191 [Mate]: SFK-N19T:34 ↔ JIS B 1176 - メートル M8 x 12:33
- メイト:192 [Mate]: SFK-N19T:34 ↔ JIS B 1176 - メートル M8 x 12:33
- メイト:193 [Mate]: SFK-N19T:34 ↔ JIS B 1176 - メートル M8 x 12:34
- メイト:194 [Mate]: SFK-N19T:34 ↔ JIS B 1176 - メートル M8 x 12:34
- メイト:195 [Mate]: SFK-N19T:29 ↔ JIS B 1176 - メートル M8 x 12:35
- メイト:196 [Mate]: SFK-N19T:29 ↔ JIS B 1176 - メートル M8 x 12:35
- メイト:197 [Mate]: SFK-N19T:29 ↔ JIS B 1176 - メートル M8 x 12:36
- メイト:198 [Mate]: SFK-N19T:29 ↔ JIS B 1176 - メートル M8 x 12:36
- メイト:199 [Mate]: SFK-N19T:30 ↔ JIS B 1176 - メートル M8 x 12:37
- メイト:200 [Mate]: SFK-N19T:30 ↔ JIS B 1176 - メートル M8 x 12:37
- メイト:201 [Mate]: SFK-N19T:30 ↔ JIS B 1176 - メートル M8 x 12:38
- メイト:202 [Mate]: SFK-N19T:30 ↔ JIS B 1176 - メートル M8 x 12:38
- 挿入:9 [Insert]: SFK-N19T:38 ↔ JIS B 1176 - メートル M8 x 12:39
- 挿入:10 [Insert]: SFK-N19T:38 ↔ JIS B 1176 - メートル M8 x 12:40
- 挿入:11 [Insert]: SFK-N19T:56 ↔ JIS B 1176 - メートル M8 x 12:41
- 挿入:12 [Insert]: SFK-N19T:56 ↔ JIS B 1176 - メートル M8 x 12:42
- メイト:203 [Mate]: SFK-N19T:43 ↔ JIS B 1176 - メートル M8 x 12:43
- メイト:204 [Mate]: SFK-N19T:43 ↔ JIS B 1176 - メートル M8 x 12:43
- メイト:205 [Mate]: SFK-N19T:43 ↔ JIS B 1176 - メートル M8 x 12:44
- メイト:206 [Mate]: SFK-N19T:43 ↔ JIS B 1176 - メートル M8 x 12:44
- メイト:207 [Mate]: SFK-N19T:43 ↔ JIS B 1176 - メートル M8 x 12:45
- メイト:208 [Mate]: SFK-N19T:43 ↔ JIS B 1176 - メートル M8 x 12:45
- メイト:209 [Mate]: SFK-N19T:43 ↔ JIS B 1176 - メートル M8 x 12:46
- メイト:210 [Mate]: SFK-N19T:43 ↔ JIS B 1176 - メートル M8 x 12:46
- メイト:211 [Mate]: SFK-N19T:44 ↔ JIS B 1176 - メートル M8 x 12:47
- メイト:212 [Mate]: SFK-N19T:44 ↔ JIS B 1176 - メートル M8 x 12:47
- メイト:213 [Mate]: SFK-N19T:44 ↔ JIS B 1176 - メートル M8 x 12:48
- メイト:214 [Mate]: SFK-N19T:44 ↔ JIS B 1176 - メートル M8 x 12:48
- 挿入:13 [Insert]: SFK-N19T:25 ↔ JIS B 1176 - メートル M8 x 12:49
- 挿入:14 [Insert]: SFK-N19T:25 ↔ JIS B 1176 - メートル M8 x 12:50
- メイト:215 [Mate]: SFK-N19T:33 ↔ JIS B 1176 - メートル M8 x 12:51
- メイト:216 [Mate]: SFK-N19T:33 ↔ JIS B 1176 - メートル M8 x 12:51
- メイト:217 [Mate]: SFK-N19T:33 ↔ JIS B 1176 - メートル M8 x 12:52
- メイト:218 [Mate]: SFK-N19T:33 ↔ JIS B 1176 - メートル M8 x 12:52
- メイト:219 [Mate]: SFK-N19T:21 ↔ JIS B 1176 - メートル M8 x 12:53
- メイト:220 [Mate]: SFK-N19T:21 ↔ JIS B 1176 - メートル M8 x 12:53
- メイト:221 [Mate]: SFK-N19T:21 ↔ JIS B 1176 - メートル M8 x 12:54
- メイト:222 [Mate]: SFK-N19T:21 ↔ JIS B 1176 - メートル M8 x 12:54
- メイト:223 [Mate]: SFK-N19T:11 ↔ JIS B 1176 - メートル M8 x 12:55
- メイト:224 [Mate]: SFK-N19T:11 ↔ JIS B 1176 - メートル M8 x 12:55
- メイト:225 [Mate]: SFK-N19T:11 ↔ JIS B 1176 - メートル M8 x 12:56
- メイト:226 [Mate]: SFK-N19T:11 ↔ JIS B 1176 - メートル M8 x 12:56
- メイト:227 [Mate]: SFK-N19T:11 ↔ JIS B 1176 - メートル M8 x 12:57
- メイト:228 [Mate]: SFK-N19T:11 ↔ JIS B 1176 - メートル M8 x 12:57